# Autodesk Inventor assembly: 膝_6_1_MIR1
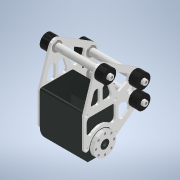
[picture p0: Inventor's stored thumbnail of the model, 180x180]
Saved by Autodesk Inventor 2020.4 (Build 244396000, 396)
## iProperties
Created: 2016-08-23
Part Number: 膝_6_1_MIR1
Material: 一般
Document SubType Name: Assembly
Designer: masato
Mass: 259.679 g
Surface Area: 513.454 cm^2
Volume: 137.54 cm^3
Density: 1.88802 g/cm^3
Author: hiro
## Documents named in this file (9)
- C:\Users\masato\Documents\Inventor\CITBrains\OpenPlatform_ver3_0\下半身_160823\膝\膝_6_1_MIR1.iam
- C:\Users\masato\Documents\Inventor\CITBrains\OpenPlatform_ver3_0\既製品\B3M11xx.ipt
- B3M11xx.ipt
- C:\Users\masato\Documents\Inventor\CITBrains\OpenPlatform_ver3_0\下半身_160823\膝\膝_メインフレーム.ipt
- C:\Users\masato\Documents\Inventor\CITBrains\OpenPlatform_ver3_0\既製品\NSK_RB_MF85ZZ\MF85ZZ.iam
- C:\Users\masato\Documents\Inventor\CITBrains\OpenPlatform_ver3_0\既製品\free_horn.ipt
- C:\Users\masato\Documents\Inventor\CITBrains\OpenPlatform_ver3_0\既製品\SSFRMHHS6-38_3-F12_7-P5-T12_7-M3-SC0-TF12_7-TT12_7.ipt
- C:\Users\masato\Documents\Inventor\CITBrains\OpenPlatform_ver3_0\既製品\CC-0513-25B.ipt
- C:\Users\masato\Documents\Inventor\CITBrains\OpenPlatform_ver3_0\既製品\CC-0513-50B.ipt
## Components (25 placed, 7 different names)
1. B3M11xx:1 — 挿入:99, 挿入:98, 挿入:97, 挿入:96, 挿入:92
2. 膝_メインフレーム:1 — 挿入:99, 挿入:98, 挿入:80, 挿入:82, 挿入:81, 挿入:103, 挿入:104, 挿入:105
3. 膝_メインフレーム:2 — 挿入:97, 挿入:96, 挿入:77, 挿入:78, 挿入:79, 挿入:106, 挿入:107, 挿入:108
4. MF85ZZ:1 [sub-assembly] — 挿入:80, 挿入:100
5. MF85ZZ:2 [sub-assembly] — 挿入:82, 挿入:102
6. MF85ZZ:3 [sub-assembly] — 挿入:81, 挿入:101
7. MF85ZZ:4 [sub-assembly] — 挿入:77
8. MF85ZZ:5 [sub-assembly] — 挿入:78
9. MF85ZZ:6 [sub-assembly] — 挿入:79
10. free_horn:1 — 挿入:92
11. SSFRMHHS6-38_3-F12_7-P5-T12_7-M3-SC0-TF12_7-TT12_7:1 — 挿入:100
12. SSFRMHHS6-38_3-F12_7-P5-T12_7-M3-SC0-TF12_7-TT12_7:2 — 挿入:101
13. SSFRMHHS6-38_3-F12_7-P5-T12_7-M3-SC0-TF12_7-TT12_7:3 — 挿入:102
14. CC-0513-25B:1 — 挿入:103, 挿入:109
15. CC-0513-25B:2 — 挿入:104, 挿入:110
16. CC-0513-25B:3 — 挿入:105, 挿入:111
17. CC-0513-25B:4 — 挿入:106, 挿入:112
18. CC-0513-25B:5 — 挿入:107, 挿入:113
19. CC-0513-25B:6 — 挿入:108, 挿入:114
20. CC-0513-50B:1 — 挿入:109
21. CC-0513-50B:2 — 挿入:110
22. CC-0513-50B:3 — 挿入:111
23. CC-0513-50B:4 — 挿入:112
24. CC-0513-50B:5 — 挿入:113
25. CC-0513-50B:6 — 挿入:114
## Relationships (26: Insert 26)
- 挿入:99 [Insert]: B3M11xx:1 ↔ 膝_メインフレーム:1
- 挿入:98 [Insert]: B3M11xx:1 ↔ 膝_メインフレーム:1
- 挿入:97 [Insert]: B3M11xx:1 ↔ 膝_メインフレーム:2
- 挿入:96 [Insert]: B3M11xx:1 ↔ 膝_メインフレーム:2
- 挿入:80 [Insert]: 膝_メインフレーム:1 ↔ MF85ZZ:1
- 挿入:82 [Insert]: 膝_メインフレーム:1 ↔ MF85ZZ:2
- 挿入:81 [Insert]: 膝_メインフレーム:1 ↔ MF85ZZ:3
- 挿入:77 [Insert]: 膝_メインフレーム:2 ↔ MF85ZZ:4
- 挿入:78 [Insert]: 膝_メインフレーム:2 ↔ MF85ZZ:5
- 挿入:79 [Insert]: 膝_メインフレーム:2 ↔ MF85ZZ:6
- 挿入:92 [Insert]: B3M11xx:1 ↔ free_horn:1
- 挿入:100 [Insert]: MF85ZZ:1 ↔ SSFRMHHS6-38_3-F12_7-P5-T12_7-M3-SC0-TF12_7-TT12_7:1
- 挿入:101 [Insert]: MF85ZZ:3 ↔ SSFRMHHS6-38_3-F12_7-P5-T12_7-M3-SC0-TF12_7-TT12_7:2
- 挿入:102 [Insert]: MF85ZZ:2 ↔ SSFRMHHS6-38_3-F12_7-P5-T12_7-M3-SC0-TF12_7-TT12_7:3
- 挿入:103 [Insert]: 膝_メインフレーム:1 ↔ CC-0513-25B:1
- 挿入:104 [Insert]: 膝_メインフレーム:1 ↔ CC-0513-25B:2
- 挿入:105 [Insert]: 膝_メインフレーム:1 ↔ CC-0513-25B:3
- 挿入:106 [Insert]: 膝_メインフレーム:2 ↔ CC-0513-25B:4
- 挿入:107 [Insert]: 膝_メインフレーム:2 ↔ CC-0513-25B:5
- 挿入:108 [Insert]: 膝_メインフレーム:2 ↔ CC-0513-25B:6
- 挿入:109 [Insert]: CC-0513-25B:1 ↔ CC-0513-50B:1
- 挿入:110 [Insert]: CC-0513-25B:2 ↔ CC-0513-50B:2
- 挿入:111 [Insert]: CC-0513-25B:3 ↔ CC-0513-50B:3
- 挿入:112 [Insert]: CC-0513-25B:4 ↔ CC-0513-50B:4
- 挿入:113 [Insert]: CC-0513-25B:5 ↔ CC-0513-50B:5
- 挿入:114 [Insert]: CC-0513-25B:6 ↔ CC-0513-50B:6
